# Autodesk Inventor assembly: Assembly_Cube_Rect_Aperture_v3
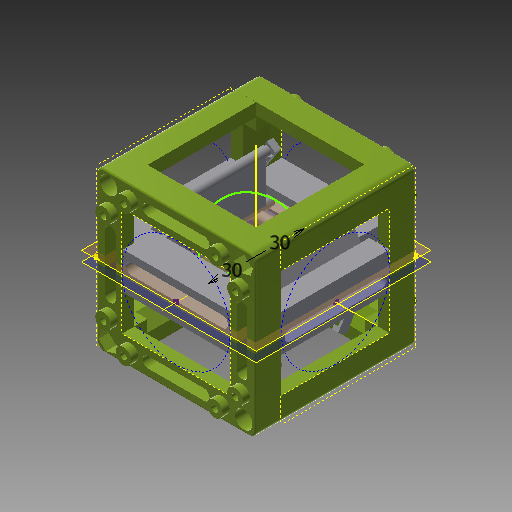
[picture p0: Inventor's stored thumbnail of the model, 512x512]
Saved by Autodesk Inventor 2019 (Build 230136000, 136)
## iProperties
Created: 2020-03-31
Part Number: Assembly_Cube_Rect_Aperture_v3
Document SubType Name: Assembly
Designer: B
Author: B
## Documents named in this file (3)
- C:\Users\marsikovabarbora\Dropbox\UC2\02_CAD\INVENTOR\uc2_v3\Assembly_Cube_Rect_Aperture_v3.iam
- C:\Users\marsikovabarbora\Dropbox\UC2\02_CAD\INVENTOR\uc2_v3\Assembly_Rect_Aperture_Insert_half.iam
- C:\Users\marsikovabarbora\Dropbox\UC2\02_CAD\INVENTOR\uc2_v3\Assembly_Cube_empty_IM_v3.iam
## Components (3 placed, 2 different names)
1. Assembly_Cube_empty_IM_v3:1 [sub-assembly] — Fluchtend:5, Fluchtend:6, Passend:3
2. Assembly_Rect_Aperture_Insert_half:1 [sub-assembly] — Fluchtend:2, Fluchtend:3, Fluchtend:4, Fluchtend:5, Passend:3
3. Assembly_Rect_Aperture_Insert_half:2 [sub-assembly] — Fluchtend:2, Fluchtend:3, Fluchtend:4, Fluchtend:6
## Relationships (9: Flush 6, Mate 3)
- [Mate]: Assembly_Cube_empty_IM_v3:1
- [Mate]: Assembly_Cube_empty_IM_v3:1
- [Flush]: Assembly_Cube_empty_IM_v3:1
- Fluchtend:2 [Flush]: Assembly_Rect_Aperture_Insert_half:1 ↔ Assembly_Rect_Aperture_Insert_half:2
- Fluchtend:3 [Flush]: Assembly_Rect_Aperture_Insert_half:1 ↔ Assembly_Rect_Aperture_Insert_half:2
- Fluchtend:4 [Flush]: Assembly_Rect_Aperture_Insert_half:1 ↔ Assembly_Rect_Aperture_Insert_half:2
- Fluchtend:5 [Flush]: Assembly_Cube_empty_IM_v3:1 ↔ Assembly_Rect_Aperture_Insert_half:1
- Fluchtend:6 [Flush]: Assembly_Cube_empty_IM_v3:1 ↔ Assembly_Rect_Aperture_Insert_half:2
- Passend:3 [Mate]: Assembly_Cube_empty_IM_v3:1 ↔ Assembly_Rect_Aperture_Insert_half:1
